# Autodesk Inventor assembly: Sessao9__08_04_2025_999_0001
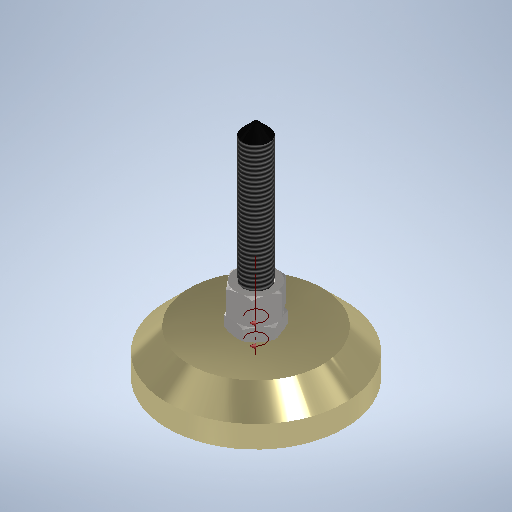
[picture p0: Inventor's stored thumbnail of the model, 512x512]
Saved by Autodesk Inventor 2025.2 (Build 292293000, 293)
## iProperties
Created: 2025-04-08
Part Number: Sessao9__08_04_2025_999_0001
Document SubType Name: Assembly
Designer: Gustavo Sousa
Author: Gustavo Sousa
## Documents named in this file (5)
- C:\Users\lucas\OneDrive\Documentos\Documentos\Gustavo\Mozangao\Robotica_Fundamentos\Inventor\Sessao9__08_04_2025\Sessao9__08_04_2025_999_0001.iam
- C:\Users\lucas\OneDrive\Documentos\Documentos\Gustavo\Mozangao\Robotica_Fundamentos\Inventor\Sessao9__08_04_2025\Sessao9__08_04_2025_0001_001.ipt
- C:\Users\lucas\OneDrive\Documentos\Documentos\Gustavo\Mozangao\Robotica_Fundamentos\Inventor\Sessao9__08_04_2025\Sessao9__08_04_2025_0002_001.ipt
- C:\Users\lucas\OneDrive\Documentos\Inventor\Content Center Files\R2025\pt-BR\ANSI B18.2.4.5M\ANSI B18.2.4.5M - M12 x 1.75.ipt
- C:\Users\lucas\OneDrive\Documentos\Inventor\Content Center Files\R2025\pt-BR\ANSI B 18.2.4.1 M(1)\ANSI B 18.2.4.1 M - M12 x 1,75Style 2.ipt
## Components (4 placed, 4 different names)
1. Sessao9__08_04_2025_0001_001:1 — Alinhado:1, Alinhado:2, Alinhado:3, Coincidente:2, Coincidente:4, Alinhado:4
2. Sessao9__08_04_2025_0002_001:1 — Coincidente:1, Coincidente:2, Coincidente:3, Coincidente:5, Alinhado:5
3. Contraporca sextavada - Métrica M12 x 1.75:1 — Coincidente:3, Coincidente:4, Coincidente:6
4. Porca sextavada Métrica M12 x 1,75:1 — Coincidente:5, Coincidente:6
## Relationships (11: Mate 6, Flush 5)
- Alinhado:1 [Flush]: Sessao9__08_04_2025_0001_001:1
- Alinhado:2 [Flush]: Sessao9__08_04_2025_0001_001:1
- Alinhado:3 [Flush]: Sessao9__08_04_2025_0001_001:1
- Coincidente:1 [Mate]: Sessao9__08_04_2025_0002_001:1
- Coincidente:2 [Mate]: Sessao9__08_04_2025_0001_001:1 ↔ Sessao9__08_04_2025_0002_001:1
- Coincidente:3 [Mate]: Sessao9__08_04_2025_0002_001:1 ↔ Contraporca sextavada - Métrica M12 x 1.75:1
- Coincidente:4 [Mate]: Sessao9__08_04_2025_0001_001:1 ↔ Contraporca sextavada - Métrica M12 x 1.75:1
- Coincidente:5 [Mate]: Sessao9__08_04_2025_0002_001:1 ↔ Porca sextavada Métrica M12 x 1,75:1
- Coincidente:6 [Mate]: Contraporca sextavada - Métrica M12 x 1.75:1 ↔ Porca sextavada Métrica M12 x 1,75:1
- Alinhado:4 [Flush]: Sessao9__08_04_2025_0001_001:1
- Alinhado:5 [Flush]: Sessao9__08_04_2025_0002_001:1
